# Autodesk Inventor assembly: Ninja cylinder thing
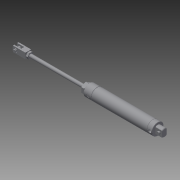
[picture p0: Inventor's stored thumbnail of the model, 180x180]
Saved by Autodesk Inventor 2013 (Build 170138000, 138)
## iProperties
Created: 2013-03-16
Part Number: Ninja cylinder thing
Document SubType Name: Assembly
Designer: Arpan
Author: Arpan
## Documents named in this file (10)
- C:\Users\Arpan\Documents\GitHub\frc2013CAD\Ninja cylinder thing.iam
- C:\Users\Arpan\Downloads\PARTserver55657037\Imported Components\176_DP_D_229__F_D_231_1__F_D_3556__2_03\1.ipt
- C:\Users\Arpan\Downloads\PARTserver55657037\Imported Components\176_DP_D_229__F_D_231_1__F_D_3556__2_03\2.ipt
- C:\Users\Arpan\Downloads\PARTserver55657037\Imported Components\176_DP_D_229__F_D_231_1__F_D_3556__2_03\3.ipt
- C:\Users\Arpan\Downloads\PARTserver55657037\Imported Components\176_DP_D_229__F_D_231_1__F_D_3556__2_03\4.ipt
- C:\Users\Arpan\Downloads\PARTserver55657037\Imported Components\176_DP_D_229__F_D_231_1__F_D_3556__2_03\7.ipt
- C:\Users\Arpan\Downloads\PARTserver55657037\Imported Components\176_DP_D_229__F_D_231_1__F_D_3556__2_03\8.ipt
- C:\Users\Arpan\Downloads\PARTserver55657037\Imported Components\176_DP_D_229__F_D_231_1__F_D_3556__2_03\9.ipt
- C:\Users\Arpan\Downloads\PARTserver55657037\Imported Components\176_DP_D_229__F_D_231_1__F_D_3556__2_03\10.ipt
- C:\Users\Arpan\Downloads\PARTserver55657037\Imported Components\176_DP_D_229__F_D_231_1__F_D_3556__2_03\13.ipt
## Components (9 placed, 9 different names)
1. 1:1 — Mate:3, Mate:5
2. 2:1 — Mate:1, Mate:4
3. 3:1 — Mate:4, Angle:1
4. 4:1
5. 7:1
6. 8:1 — Mate:1, Mate:2, Mate:3, Mate:5, Mate:7
7. 9:1 — Mate:2, Mate:6, Angle:1
8. 10:1 — Mate:6
9. 13:1 — Mate:7
## Relationships (8: Mate 7, Angle 1)
- Mate:1: 2:1 ↔ 8:1
- Mate:2: 8:1 ↔ 9:1
- Mate:3: 1:1 ↔ 8:1
- Mate:4: 2:1 ↔ 3:1
- Mate:5: 1:1 ↔ 8:1
- Mate:6: 9:1 ↔ 10:1
- Mate:7: 8:1 ↔ 13:1
- Angle:1 (0 deg): 3:1 ↔ 9:1
